# Autodesk Inventor assembly: 客户模型 M3508减速箱 减比268：17
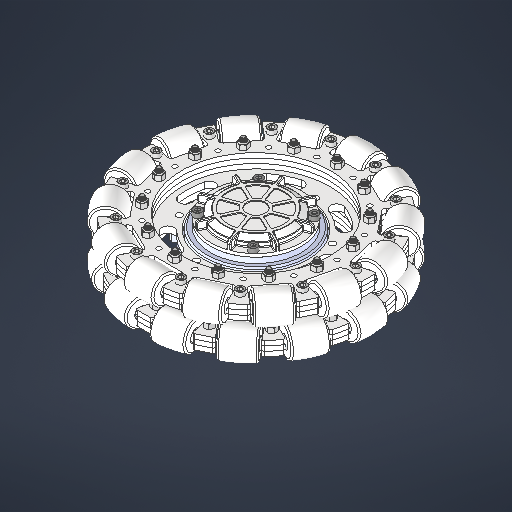
[picture p0: Inventor's stored thumbnail of the model, 512x512]
Saved by Autodesk Inventor 2025 (Build 290162000, 162)
## iProperties
Created: 2024-05-13
Part Number: 客户模型 M3508减速箱 减比268：17
Description: STEP AP214
Document SubType Name: Assembly
Designer: HZD
Sending System: SolidWorks 2021
Preprocessor: SwSTEP 2.0
Title: ¿Í»§Ä£ÐÍ M3508¼õËÙÏä ¼õ±È268£º17.STEP
Revision Number: ÈÎºÎ
## Documents named in this file (4)
- C:\1A_Engineering_files\RCInventor并联腿\铝件版本\轮系\客户模型 M3508减速箱 减比268：17.iam
- C:\1A_Engineering_files\RCInventor并联腿\铝件版本\轮系\¿Í»§Ä£ÐÍ M3508¼õËÙÏä ¼õ±È268£º17.0004.ipt
- C:\1A_Engineering_files\RCInventor并联腿\铝件版本\轮系\OTOW-全向轮连轴板-上交联轴器1.ipt
- C:\1A_Engineering_files\RCInventor并联腿\铝件版本\轮系\OTOW-全向轮装配.ipt
## Components (3 placed, 3 different names)
1. ¿Í»§Ä£ÐÍ M3508¼õËÙÏä ¼õ±È268£º17_1 — 配合:1, 配合:2, 配合:3
2. OTOW-全向轮连轴板-上交联轴器1:1 — 配合:1, 配合:2, 配合:3, 配合:4, 配合:5
3. OTOW-全向轮装配:1 — 配合:4, 配合:5
## Relationships (5: Mate 5)
- 配合:1 [Mate]: ¿Í»§Ä£ÐÍ M3508¼õËÙÏä ¼õ±È268£º17_1 ↔ OTOW-全向轮连轴板-上交联轴器1:1
- 配合:2 [Mate]: ¿Í»§Ä£ÐÍ M3508¼õËÙÏä ¼õ±È268£º17_1 ↔ OTOW-全向轮连轴板-上交联轴器1:1
- 配合:3 [Mate]: ¿Í»§Ä£ÐÍ M3508¼õËÙÏä ¼õ±È268£º17_1 ↔ OTOW-全向轮连轴板-上交联轴器1:1
- 配合:4 [Mate]: OTOW-全向轮连轴板-上交联轴器1:1 ↔ OTOW-全向轮装配:1
- 配合:5 [Mate]: OTOW-全向轮连轴板-上交联轴器1:1 ↔ OTOW-全向轮装配:1
